# Autodesk Inventor assembly: LS Conveyor Axle
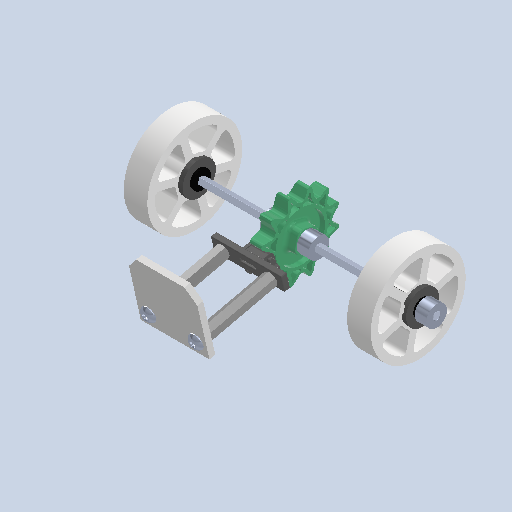
[picture p0: Inventor's stored thumbnail of the model, 512x512]
Saved by Autodesk Inventor 2025.1 (Build 291241020, 241B)
## iProperties
Created: 2024-12-19
Part Number: LS Conveyor Axle
Document SubType Name: Assembly
Designer: Juan
Author: Juan
## Documents named in this file (14)
- C:\Users\AtuStem\Documents\GitHub\ATUM-V5RC-High-Stakes-CAD\Robot\Subassemblies\LS Conveyor Axle.iam
- C:\Users\AtuStem\Documents\GitHub\ATUM-V5RC-High-Stakes-CAD\VEX-CAD-Inventor\Motion\Sprockets\9P Sprocket\9P 12T Sprocket, Square.iam
- C:\Users\Juan\Documents\GitHub\ATUM-VRC-High-Stakes-CAD\VEX-CAD-Inventor\Motion\Sprockets\9P Sprocket.iam
- C:\Users\AtuStem\Documents\GitHub\ATUM-V5RC-High-Stakes-CAD\VEX-CAD-Inventor\Motion\Chain 9P\Chain Attachment Link.ipt
- C:\Users\AtuStem\Documents\GitHub\ATUM-V5RC-High-Stakes-CAD\Hook.ipt
- C:\Users\AtuStem\Documents\GitHub\ATUM-V5RC-High-Stakes-CAD\VEX-CAD-Inventor\Structure\Standoff\Standoff 1.50.ipt
- C:\Users\Juan\Documents\GitHub\ATUM-VRC-High-Stakes-CAD\VEX-CAD-Inventor\Structure\Standoff.ipt
- C:\Users\Juan\Documents\GitHub\ATUM-VRC-High-Stakes-CAD\VEX-CAD-Inventor\Motion\Shaft LS\Shaft LS.ipt
- C:\Users\AtuStem\Documents\GitHub\ATUM-V5RC-High-Stakes-CAD\VEX-CAD-Inventor\Motion\Shaft LS\Shaft Collar Metal\Shaft Collar No Screw.ipt
- C:\Users\AtuStem\Documents\GitHub\ATUM-V5RC-High-Stakes-CAD\VEX-CAD-Inventor\Motion\Insert Square.ipt
- C:\Users\AtuStem\Documents\GitHub\ATUM-V5RC-High-Stakes-CAD\Robot\Subassemblies\2.0 Flex Wheel with Insert.iam
- C:\Users\AtuStem\Documents\GitHub\ATUM-V5RC-High-Stakes-CAD\VEX-CAD-Inventor\Structure\Hardware\Screw Steel - Star\SScrew Star Smooth .375.ipt
- C:\Users\Juan\Documents\GitHub\ATUM-VRC-High-Stakes-CAD\VEX-CAD-Inventor\Structure\Hardware\Screw Steel - Star.ipt
- C:\Users\AtuStem\Documents\GitHub\ATUM-V5RC-High-Stakes-CAD\VEX-CAD-Inventor\Motion\Shaft LS\Shaft LS\Shaft LS 6.0.ipt
## Components (18 placed, 9 different names)
1. 9P 12T Sprocket, Square:1 [sub-assembly]
2. Chain Attachment Link:1
3. Hook:1 — Rigid:1, Rigid:2
4. Standoff 1.50:1
5. Standoff 1.50:2
6. Shaft LS 6.0:1 — Mate:38
7. Shaft Collar No Screw:1 — Mate:38, Mate:39
8. Shaft Collar No Screw:2
9. Insert Square:1
10. Insert Square:2 — Mate:39
11. Insert Square:3
12. Insert Square:4
13. Shaft Collar No Screw:5
14. Shaft Collar No Screw:6
15. 2.0 Flex Wheel with Insert:1 [sub-assembly]
16. 2.0 Flex Wheel with Insert:2 [sub-assembly]
17. SScrew Star Smooth .375:1 — Rigid:1
18. SScrew Star Smooth .375:2 — Rigid:2
## Relationships (44: Mate 36, Angle 4, Flush 2, WeldJoint 2)
- [Mate]: 9P 12T Sprocket, Square:1 ↔ Chain Attachment Link:1
- [Mate] (-2.54 mm): 9P 12T Sprocket, Square:1 ↔ Chain Attachment Link:1
- [Mate]: Chain Attachment Link:1 ↔ Standoff 1.50:1
- [Mate]: Chain Attachment Link:1 ↔ Standoff 1.50:2
- [Mate]: Chain Attachment Link:1 ↔ Standoff 1.50:2
- [Mate] (0.1524 mm): 9P 12T Sprocket, Square:1 ↔ Chain Attachment Link:1
- [Mate]: Chain Attachment Link:1 ↔ Standoff 1.50:1
- [Mate]: Hook:1 ↔ Standoff 1.50:1
- [Mate]: Hook:1 ↔ Standoff 1.50:2
- [Mate]: Hook:1 ↔ Standoff 1.50:2
- [Mate]: 9P 12T Sprocket, Square:1 ↔ Shaft LS 6.0:1
- [Mate]: 9P 12T Sprocket, Square:1 ↔ Shaft LS 6.0:1
- [Mate]: 9P 12T Sprocket, Square:1 ↔ Shaft Collar No Screw:1
- [Mate]: 9P 12T Sprocket, Square:1 ↔ Shaft Collar No Screw:2
- [Angle] (0 deg): Shaft LS 6.0:1 ↔ Shaft Collar No Screw:1
- [Angle] (0 deg): Shaft LS 6.0:1 ↔ Shaft Collar No Screw:2
- [Mate]: Insert Square:1 ↔ 2.0 Flex Wheel with Insert:1
- [Mate]: Insert Square:1 ↔ 2.0 Flex Wheel with Insert:1
- [Mate]: Insert Square:2 ↔ 2.0 Flex Wheel with Insert:1
- [Mate]: Insert Square:2 ↔ 2.0 Flex Wheel with Insert:1
- [Mate]: Insert Square:3 ↔ 2.0 Flex Wheel with Insert:2
- [Mate]: Insert Square:3 ↔ 2.0 Flex Wheel with Insert:2
- [Mate]: Insert Square:4 ↔ 2.0 Flex Wheel with Insert:2
- [Mate]: Insert Square:4 ↔ 2.0 Flex Wheel with Insert:2
- [Mate]: Insert Square:3 ↔ 2.0 Flex Wheel with Insert:2
- [Mate]: Insert Square:4 ↔ 2.0 Flex Wheel with Insert:2
- [Mate]: Insert Square:1 ↔ 2.0 Flex Wheel with Insert:1
- [Mate]: Insert Square:2 ↔ 2.0 Flex Wheel with Insert:1
- [Mate]: Shaft LS 6.0:1 ↔ Insert Square:1
- [Mate]: Shaft LS 6.0:1 ↔ Insert Square:1
- [Mate]: Shaft LS 6.0:1 ↔ Insert Square:4
- [Mate]: Shaft LS 6.0:1 ↔ Insert Square:4
- [Mate]: Insert Square:1 ↔ Shaft Collar No Screw:5
- [Angle] (0 deg): Shaft LS 6.0:1 ↔ Shaft Collar No Screw:5
- [Mate]: Insert Square:4 ↔ Shaft Collar No Screw:6
- [Angle] (0 deg): Shaft LS 6.0:1 ↔ Shaft Collar No Screw:6
- [Mate]: Insert Square:4 ↔ Shaft Collar No Screw:6
- [Mate]: Insert Square:1 ↔ Shaft Collar No Screw:5
- [Flush]: Shaft LS 6.0:1 ↔ Shaft Collar No Screw:6
- [Flush]: Shaft LS 6.0:1 ↔ Shaft Collar No Screw:5
- Rigid:1 [WeldJoint]: Hook:1 ↔ SScrew Star Smooth .375:1
- Rigid:2 [WeldJoint]: Hook:1 ↔ SScrew Star Smooth .375:2
- Mate:38: Shaft LS 6.0:1 ↔ Shaft Collar No Screw:1
- Mate:39 (36.8554 mm): Shaft Collar No Screw:1 ↔ Insert Square:2
## Named parameters: d1540_d1536 = 0 mm, d1541_d1537 = 0 mm, d1542_d1538 = 0 mm, d1543_d1539 = 0 mm
